# Autodesk Inventor assembly: upper_arm_link
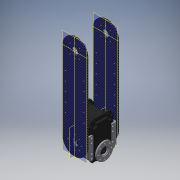
[picture p0: Inventor's stored thumbnail of the model, 180x180]
Saved by Autodesk Inventor 2018 (Build 220112000, 112)
## iProperties
Created: 2018-12-01
Part Number: upper_arm_link
Document SubType Name: Assembly
Designer: jaspe
Author: jaspe
## Documents named in this file (4)
- C:\Users\jaspe\bitbots_hardware\wolfgang\assembly\arms\upper_arm_link.iam
- C:\Users\jaspe\bitbots_hardware\wolfgang\assembly\arms\upperarm.ipt
- C:\Users\jaspe\bitbots_hardware\wolfgang\assembly\motors\MX64\Mx64_with_bearing.iam
- C:\Users\jaspe\bitbots_hardware\wolfgang\assembly\arms\connector_shoulder.ipt
## Components (5 placed, 3 different names)
1. upperarm:1 — Mate:13, Mate:14
2. upperarm:2 — Mate:14
3. Mx64_with_bearing:1 [sub-assembly] — Flush:1, Mate:12, Angle:1
4. connector_shoulder:1
5. connector_shoulder:2 — Mate:13
## Relationships (16: Mate 14, Flush 1, Angle 1)
- [Mate]: Mx64_with_bearing:1 ↔ connector_shoulder:2
- [Mate]: Mx64_with_bearing:1 ↔ connector_shoulder:2
- [Mate]: Mx64_with_bearing:1 ↔ connector_shoulder:2
- [Mate]: Mx64_with_bearing:1 ↔ connector_shoulder:1
- [Mate]: Mx64_with_bearing:1 ↔ connector_shoulder:1
- [Mate]: Mx64_with_bearing:1 ↔ connector_shoulder:1
- [Mate]: upperarm:2 ↔ connector_shoulder:1
- [Mate]: upperarm:2 ↔ connector_shoulder:1
- [Mate]: upperarm:2 ↔ connector_shoulder:1
- [Mate]: upperarm:1 ↔ connector_shoulder:2
- Flush:1 (-20.5 mm): Mx64_with_bearing:1
- Mate:11
- Mate:12: Mx64_with_bearing:1
- Mate:13: upperarm:1 ↔ connector_shoulder:2
- Angle:1 (0 deg): Mx64_with_bearing:1
- Mate:14: upperarm:1 ↔ upperarm:2
